# Autodesk Inventor assembly: клешня сбока
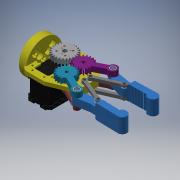
[picture p0: Inventor's stored thumbnail of the model, 180x180]
Saved by Autodesk Inventor 2019 (Build 230136000, 136)
## iProperties
Created: 2019-08-18
Part Number: клешня сбока
Material: Типовые
Document SubType Name: Assembly
Designer: Петров Иван
Mass: 103.83 g
Surface Area: 471.759 cm^2
Volume: 98.2815 cm^3
Density: 1.05645 g/cm^3
Author: Петров Иван
## Documents named in this file (10)
- E:\IVAN\Ivan_desktop\Kvantorium\Projects\optimal_gripper\hardware\КВ33.044.200 - Сборка зажима.iam
- E:\IVAN\Ivan_desktop\Kvantorium\Projects\optimal_gripper\hardware\КВ33.044.201 - Опора зажимного механизма.ipt
- E:\IVAN\Ivan_desktop\Kvantorium\Projects\optimal_gripper\hardware\Стандартные изделия\Сервомотор Dynamixel AX-12A\AX-12.iam
- E:\IVAN\Ivan_desktop\Kvantorium\Projects\optimal_gripper\hardware\Стандартные изделия\Подшипник 4x8x3.ipt
- E:\IVAN\Ivan_desktop\Kvantorium\Projects\optimal_gripper\hardware\КВ33.044.102 - Колесо зубчатое сервомотора.ipt
- E:\IVAN\Ivan_desktop\Kvantorium\Projects\optimal_gripper\hardware\КВ33.044.205 - Рычаг приводной 17 зубьев.ipt
- E:\IVAN\Ivan_desktop\Kvantorium\Projects\optimal_gripper\hardware\КВ33.044.206 - Рычаг приводной 16 зубьев.ipt
- E:\IVAN\Ivan_desktop\Kvantorium\Projects\optimal_gripper\hardware\КВ33.044.202 -Прихват.ipt
- E:\IVAN\Ivan_desktop\Kvantorium\Projects\optimal_gripper\hardware\КВ33.044.203 - Рычаг толстый.ipt
- E:\IVAN\Ivan_desktop\Kvantorium\Projects\optimal_gripper\hardware\КВ33.044.204 -Рычаг тонкий.ipt
## Components (36 placed, 9 different names)
1. КВ33.044.201 - Опора зажимного механизма:1 — Совмещение:40, Совмещение:42, Совмещение:50, Совмещение:51, Совмещение:52, Совмещение:53, Совмещение:54, Совмещение:55, Совмещение:56, Совмещение:57, Совмещение:58, Совмещение:61, Совмещение:62, Совмещение:63, Совмещение:64, Совмещение:65, Совмещение:66, Совмещение:67, Совмещение:68, Совмещение:73, Совмещение:75, Совмещение:84, Совмещение:87, Совмещение:126, Совмещение:129, Совмещение:132, Совмещение:135
2. AX-12:1 [sub-assembly] — Совмещение:40, Совмещение:42, Совмещение:50, Совмещение:59, Совмещение:60
3. Подшипник 4x8x3:1 — Совмещение:53, Совмещение:54, Совмещение:85
4. Подшипник 4x8x3:2 — Совмещение:55, Совмещение:56, Совмещение:130
5. Подшипник 4x8x3:3 — Совмещение:51, Совмещение:52, Совмещение:86
6. Подшипник 4x8x3:4 — Совмещение:57, Совмещение:58, Совмещение:127
7. КВ33.044.102 - Колесо зубчатое сервомотора:1 — Совмещение:59, Совмещение:60, Направление навивки:1
8. КВ33.044.205 - Рычаг приводной 17 зубьев:1 — Совмещение:69, Совмещение:70, Совмещение:76, Совмещение:102, Совмещение:103, Совмещение:106, Совмещение:107, Совмещение:123, Направление навивки:1, Направление навивки:2
9. КВ33.044.206 - Рычаг приводной 16 зубьев:1 — Совмещение:71, Совмещение:72, Совмещение:74, Совмещение:88, Совмещение:99, Совмещение:100, Совмещение:101, Совмещение:104, Совмещение:105, Совмещение:108, Совмещение:109, Направление навивки:2
10. Подшипник 4x8x3:5 — Совмещение:61, Совмещение:62, Совмещение:74
11. Подшипник 4x8x3:6 — Совмещение:63, Совмещение:64, Совмещение:76
12. Подшипник 4x8x3:8 — Совмещение:65, Совмещение:66, Совмещение:133
13. Подшипник 4x8x3:9 — Совмещение:67, Совмещение:68, Совмещение:136
14. Подшипник 4x8x3:10 — Совмещение:69, Совмещение:70, Совмещение:75
15. Подшипник 4x8x3:11 — Совмещение:71, Совмещение:72, Совмещение:73
16. КВ33.044.203 - Рычаг толстый:2 — Совмещение:84, Совмещение:85, Совмещение:125
17. КВ33.044.203 - Рычаг толстый:3 — Совмещение:86, Совмещение:87, Совмещение:110
18. КВ33.044.202 -Прихват:1 — Совмещение:88, Совмещение:91, Совмещение:92, Совмещение:93, Совмещение:94, Совмещение:95, Совмещение:96, Совмещение:97, Совмещение:98, Совмещение:99, Совмещение:108, Совмещение:109
19. КВ33.044.204 -Рычаг тонкий:1 — Совмещение:126, Совмещение:127, Совмещение:128
20. КВ33.044.204 -Рычаг тонкий:2 — Совмещение:129, Совмещение:130, Совмещение:131
21. КВ33.044.204 -Рычаг тонкий:3 — Совмещение:132, Совмещение:133, Совмещение:134
22. КВ33.044.204 -Рычаг тонкий:4 — Совмещение:135, Совмещение:136, Совмещение:137
23. Подшипник 4x8x3:12 — Совмещение:97, Совмещение:98
24. Подшипник 4x8x3:13 — Совмещение:95, Совмещение:96, Совмещение:137
25. Подшипник 4x8x3:14 — Совмещение:93, Совмещение:94, Совмещение:128
26. Подшипник 4x8x3:15 — Совмещение:91, Совмещение:92, Совмещение:110
27. Подшипник 4x8x3:16 — Совмещение:100, Совмещение:101
28. Подшипник 4x8x3:17 — Совмещение:102, Совмещение:103, Совмещение:124
29. Подшипник 4x8x3:18 — Совмещение:106, Совмещение:107
30. Подшипник 4x8x3:19 — Совмещение:104, Совмещение:105
31. КВ33.044.202 -Прихват:2 — Совмещение:119, Совмещение:120, Совмещение:121, Совмещение:122, Совмещение:123
32. Подшипник 4x8x3:20 — Совмещение:124, Совмещение:125
33. Подшипник 4x8x3:21 — Совмещение:120
34. Подшипник 4x8x3:22 — Совмещение:119, Совмещение:131
35. Подшипник 4x8x3:23
36. Подшипник 4x8x3:24 — Совмещение:121, Совмещение:122, Совмещение:134
## Relationships (82: Mate 80, RelateRotation 2)
- Совмещение:40 [Mate]: КВ33.044.201 - Опора зажимного механизма:1 ↔ AX-12:1
- Совмещение:42 [Mate]: КВ33.044.201 - Опора зажимного механизма:1 ↔ AX-12:1
- Совмещение:50 [Mate]: КВ33.044.201 - Опора зажимного механизма:1 ↔ AX-12:1
- Совмещение:51 [Mate]: КВ33.044.201 - Опора зажимного механизма:1 ↔ Подшипник 4x8x3:3
- Совмещение:52 [Mate]: КВ33.044.201 - Опора зажимного механизма:1 ↔ Подшипник 4x8x3:3
- Совмещение:53 [Mate]: КВ33.044.201 - Опора зажимного механизма:1 ↔ Подшипник 4x8x3:1
- Совмещение:54 [Mate]: КВ33.044.201 - Опора зажимного механизма:1 ↔ Подшипник 4x8x3:1
- Совмещение:55 [Mate]: КВ33.044.201 - Опора зажимного механизма:1 ↔ Подшипник 4x8x3:2
- Совмещение:56 [Mate]: КВ33.044.201 - Опора зажимного механизма:1 ↔ Подшипник 4x8x3:2
- Совмещение:57 [Mate]: КВ33.044.201 - Опора зажимного механизма:1 ↔ Подшипник 4x8x3:4
- Совмещение:58 [Mate]: КВ33.044.201 - Опора зажимного механизма:1 ↔ Подшипник 4x8x3:4
- Совмещение:59 [Mate]: AX-12:1 ↔ КВ33.044.102 - Колесо зубчатое сервомотора:1
- Совмещение:60 [Mate]: AX-12:1 ↔ КВ33.044.102 - Колесо зубчатое сервомотора:1
- Совмещение:61 [Mate]: КВ33.044.201 - Опора зажимного механизма:1 ↔ Подшипник 4x8x3:5
- Совмещение:62 [Mate]: КВ33.044.201 - Опора зажимного механизма:1 ↔ Подшипник 4x8x3:5
- Совмещение:63 [Mate]: КВ33.044.201 - Опора зажимного механизма:1 ↔ Подшипник 4x8x3:6
- Совмещение:64 [Mate]: КВ33.044.201 - Опора зажимного механизма:1 ↔ Подшипник 4x8x3:6
- Совмещение:65 [Mate]: КВ33.044.201 - Опора зажимного механизма:1 ↔ Подшипник 4x8x3:8
- Совмещение:66 [Mate]: КВ33.044.201 - Опора зажимного механизма:1 ↔ Подшипник 4x8x3:8
- Совмещение:67 [Mate]: КВ33.044.201 - Опора зажимного механизма:1 ↔ Подшипник 4x8x3:9
- Совмещение:68 [Mate]: КВ33.044.201 - Опора зажимного механизма:1 ↔ Подшипник 4x8x3:9
- Совмещение:69 [Mate]: КВ33.044.205 - Рычаг приводной 17 зубьев:1 ↔ Подшипник 4x8x3:10
- Совмещение:70 [Mate]: КВ33.044.205 - Рычаг приводной 17 зубьев:1 ↔ Подшипник 4x8x3:10
- Совмещение:71 [Mate]: КВ33.044.206 - Рычаг приводной 16 зубьев:1 ↔ Подшипник 4x8x3:11
- Совмещение:72 [Mate]: КВ33.044.206 - Рычаг приводной 16 зубьев:1 ↔ Подшипник 4x8x3:11
- Совмещение:73 [Mate]: КВ33.044.201 - Опора зажимного механизма:1 ↔ Подшипник 4x8x3:11
- Совмещение:74 [Mate]: КВ33.044.206 - Рычаг приводной 16 зубьев:1 ↔ Подшипник 4x8x3:5
- Совмещение:75 [Mate]: КВ33.044.201 - Опора зажимного механизма:1 ↔ Подшипник 4x8x3:10
- Совмещение:76 [Mate]: КВ33.044.205 - Рычаг приводной 17 зубьев:1 ↔ Подшипник 4x8x3:6
- Совмещение:84 [Mate]: КВ33.044.201 - Опора зажимного механизма:1 ↔ КВ33.044.203 - Рычаг толстый:2
- Совмещение:85 [Mate]: Подшипник 4x8x3:1 ↔ КВ33.044.203 - Рычаг толстый:2
- Совмещение:86 [Mate]: Подшипник 4x8x3:3 ↔ КВ33.044.203 - Рычаг толстый:3
- Совмещение:87 [Mate]: КВ33.044.201 - Опора зажимного механизма:1 ↔ КВ33.044.203 - Рычаг толстый:3
- Совмещение:88 [Mate]: КВ33.044.206 - Рычаг приводной 16 зубьев:1 ↔ КВ33.044.202 -Прихват:1
- Совмещение:91 [Mate]: КВ33.044.202 -Прихват:1 ↔ Подшипник 4x8x3:15
- Совмещение:92 [Mate]: КВ33.044.202 -Прихват:1 ↔ Подшипник 4x8x3:15
- Совмещение:93 [Mate]: КВ33.044.202 -Прихват:1 ↔ Подшипник 4x8x3:14
- Совмещение:94 [Mate]: КВ33.044.202 -Прихват:1 ↔ Подшипник 4x8x3:14
- Совмещение:95 [Mate]: КВ33.044.202 -Прихват:1 ↔ Подшипник 4x8x3:13
- Совмещение:96 [Mate]: КВ33.044.202 -Прихват:1 ↔ Подшипник 4x8x3:13
- Совмещение:97 [Mate]: КВ33.044.202 -Прихват:1 ↔ Подшипник 4x8x3:12
- Совмещение:98 [Mate]: КВ33.044.202 -Прихват:1 ↔ Подшипник 4x8x3:12
- Совмещение:99 [Mate]: КВ33.044.206 - Рычаг приводной 16 зубьев:1 ↔ КВ33.044.202 -Прихват:1
- Совмещение:100 [Mate]: КВ33.044.206 - Рычаг приводной 16 зубьев:1 ↔ Подшипник 4x8x3:16
- Совмещение:101 [Mate]: КВ33.044.206 - Рычаг приводной 16 зубьев:1 ↔ Подшипник 4x8x3:16
- Совмещение:102 [Mate]: КВ33.044.205 - Рычаг приводной 17 зубьев:1 ↔ Подшипник 4x8x3:17
- Совмещение:103 [Mate]: КВ33.044.205 - Рычаг приводной 17 зубьев:1 ↔ Подшипник 4x8x3:17
- Совмещение:104 [Mate]: КВ33.044.206 - Рычаг приводной 16 зубьев:1 ↔ Подшипник 4x8x3:19
- Совмещение:105 [Mate]: КВ33.044.206 - Рычаг приводной 16 зубьев:1 ↔ Подшипник 4x8x3:19
- Совмещение:106 [Mate]: КВ33.044.205 - Рычаг приводной 17 зубьев:1 ↔ Подшипник 4x8x3:18
- Совмещение:107 [Mate]: КВ33.044.205 - Рычаг приводной 17 зубьев:1 ↔ Подшипник 4x8x3:18
- Совмещение:108 [Mate]: КВ33.044.206 - Рычаг приводной 16 зубьев:1 ↔ КВ33.044.202 -Прихват:1
- Совмещение:109 [Mate]: КВ33.044.206 - Рычаг приводной 16 зубьев:1 ↔ КВ33.044.202 -Прихват:1
- Совмещение:110 [Mate]: КВ33.044.203 - Рычаг толстый:3 ↔ Подшипник 4x8x3:15
- [Mate]: КВ33.044.202 -Прихват:2 ↔ Подшипник 4x8x3:23
- [Mate]: КВ33.044.202 -Прихват:2 ↔ Подшипник 4x8x3:23
- [Mate]: КВ33.044.202 -Прихват:2 ↔ Подшипник 4x8x3:22
- [Mate]: КВ33.044.202 -Прихват:2 ↔ Подшипник 4x8x3:21
- [Mate]: КВ33.044.202 -Прихват:2 ↔ Подшипник 4x8x3:21
- [Mate]: КВ33.044.202 -Прихват:2 ↔ Подшипник 4x8x3:20
- [Mate]: КВ33.044.202 -Прихват:2 ↔ Подшипник 4x8x3:20
- Совмещение:119 [Mate]: КВ33.044.202 -Прихват:2 ↔ Подшипник 4x8x3:22
- Совмещение:120 [Mate]: КВ33.044.202 -Прихват:2 ↔ Подшипник 4x8x3:21
- Совмещение:121 [Mate]: КВ33.044.202 -Прихват:2 ↔ Подшипник 4x8x3:24
- Совмещение:122 [Mate]: КВ33.044.202 -Прихват:2 ↔ Подшипник 4x8x3:24
- Совмещение:123 [Mate]: КВ33.044.205 - Рычаг приводной 17 зубьев:1 ↔ КВ33.044.202 -Прихват:2
- Совмещение:124 [Mate]: Подшипник 4x8x3:17 ↔ Подшипник 4x8x3:20
- Совмещение:125 [Mate]: КВ33.044.203 - Рычаг толстый:2 ↔ Подшипник 4x8x3:20
- Совмещение:126 [Mate]: КВ33.044.201 - Опора зажимного механизма:1 ↔ КВ33.044.204 -Рычаг тонкий:1
- Совмещение:127 [Mate]: Подшипник 4x8x3:4 ↔ КВ33.044.204 -Рычаг тонкий:1
- Совмещение:128 [Mate]: КВ33.044.204 -Рычаг тонкий:1 ↔ Подшипник 4x8x3:14
- Совмещение:129 [Mate]: КВ33.044.201 - Опора зажимного механизма:1 ↔ КВ33.044.204 -Рычаг тонкий:2
- Совмещение:130 [Mate]: Подшипник 4x8x3:2 ↔ КВ33.044.204 -Рычаг тонкий:2
- Совмещение:131 [Mate]: КВ33.044.204 -Рычаг тонкий:2 ↔ Подшипник 4x8x3:22
- Совмещение:132 [Mate]: КВ33.044.201 - Опора зажимного механизма:1 ↔ КВ33.044.204 -Рычаг тонкий:3
- Совмещение:133 [Mate]: Подшипник 4x8x3:8 ↔ КВ33.044.204 -Рычаг тонкий:3
- Совмещение:134 [Mate]: КВ33.044.204 -Рычаг тонкий:3 ↔ Подшипник 4x8x3:24
- Совмещение:135 [Mate]: КВ33.044.201 - Опора зажимного механизма:1 ↔ КВ33.044.204 -Рычаг тонкий:4
- Совмещение:136 [Mate]: Подшипник 4x8x3:9 ↔ КВ33.044.204 -Рычаг тонкий:4
- Совмещение:137 [Mate]: КВ33.044.204 -Рычаг тонкий:4 ↔ Подшипник 4x8x3:13
- Направление навивки:1 [RelateRotation] (1.5 ul): КВ33.044.102 - Колесо зубчатое сервомотора:1 ↔ КВ33.044.205 - Рычаг приводной 17 зубьев:1
- Направление навивки:2 [RelateRotation] (1 ul): КВ33.044.205 - Рычаг приводной 17 зубьев:1 ↔ КВ33.044.206 - Рычаг приводной 16 зубьев:1
## Named parameters: d155_d142 = 0 mm, d156_d135 = 0 mm, d157_d136 = 0 mm, d159_d138 = 0 mm, d160_d139 = 0 mm, d161_d140 = 0 mm, d162_d141 = 0 mm
